# Autodesk Inventor assembly: Hook Assembly
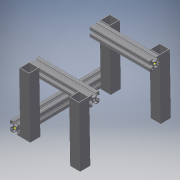
[picture p0: Inventor's stored thumbnail of the model, 180x180]
Saved by Autodesk Inventor 2018 (Build 220112000, 112)
## iProperties
Created: 2020-01-24
Part Number: Hook Assembly
Document SubType Name: Assembly
Designer: s-2513398
Author: s-2513398
## Documents named in this file (5)
- \\studenthome\students\S-2513398\Hook Files\Hook Assembly .iam
- \\studenthome\students\S-2513398\Hook Files\1010.ipt
- \\studenthome\students\S-2513398\Hook Files\Hook 1st 1x1.ipt
- \\studenthome\students\S-2513398\Hook Files\Hook 2nd 1x1.ipt
- \\studenthome\students\S-2513398\Hook Files\Hook base.ipt
## Components (7 placed, 4 different names)
1. 1010:1 — Flush:1, Flush:2, Mate:1, Flush:9, Flush:10, Mate:5
2. Hook 1st 1x1:1 — Flush:1, Flush:2, Mate:1, Flush:7, Mate:4, Flush:8
3. Hook 2nd 1x1:1 — Flush:3, Mate:2, Flush:4, Mate:3, Flush:5, Flush:6
4. Hook base:1 — Mate:3, Flush:5, Flush:6, Flush:7, Mate:4, Flush:8
5. 1010:2 — Flush:3, Mate:2, Flush:4, Mate:6, Flush:11, Flush:12
6. Hook 1st 1x1:2 — Flush:9, Flush:10, Mate:5
7. Hook 2nd 1x1:2 — Mate:6, Flush:11, Flush:12
## Relationships (18: Flush 12, Mate 6)
- Flush:1: 1010:1 ↔ Hook 1st 1x1:1
- Flush:2: 1010:1 ↔ Hook 1st 1x1:1
- Mate:1: 1010:1 ↔ Hook 1st 1x1:1
- Flush:3: Hook 2nd 1x1:1 ↔ 1010:2
- Mate:2: Hook 2nd 1x1:1 ↔ 1010:2
- Flush:4: Hook 2nd 1x1:1 ↔ 1010:2
- Mate:3: Hook 2nd 1x1:1 ↔ Hook base:1
- Flush:5: Hook 2nd 1x1:1 ↔ Hook base:1
- Flush:6: Hook 2nd 1x1:1 ↔ Hook base:1
- Flush:7: Hook 1st 1x1:1 ↔ Hook base:1
- Mate:4: Hook 1st 1x1:1 ↔ Hook base:1
- Flush:8: Hook 1st 1x1:1 ↔ Hook base:1
- Flush:9: 1010:1 ↔ Hook 1st 1x1:2
- Flush:10: 1010:1 ↔ Hook 1st 1x1:2
- Mate:5: 1010:1 ↔ Hook 1st 1x1:2
- Mate:6: 1010:2 ↔ Hook 2nd 1x1:2
- Flush:11: 1010:2 ↔ Hook 2nd 1x1:2
- Flush:12: 1010:2 ↔ Hook 2nd 1x1:2
